# Autodesk Inventor assembly: a shock cartridge
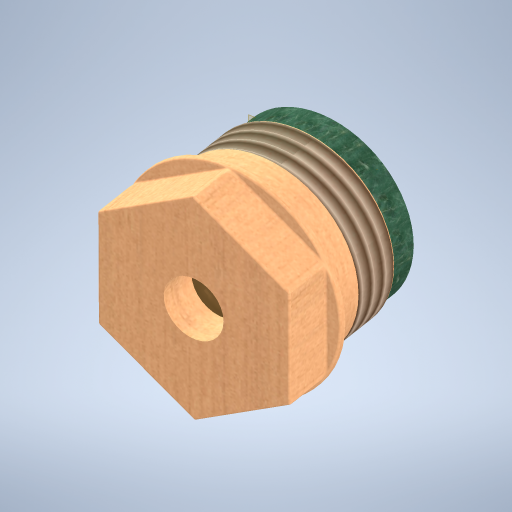
[picture p0: Inventor's stored thumbnail of the model, 512x512]
Saved by Autodesk Inventor 2024 (Build 280153000, 153)
## iProperties
Created: 2023-07-07
Part Number: a shock cartridge
Document SubType Name: Assembly
Designer: birud
Author: birud
## Documents named in this file (5)
- C:\Users\birud\OneDrive\Desktop\Openers\a shock cartridge.iam
- C:\Users\birud\OneDrive\Desktop\Openers\SA Shock Cartridge.ipt
- C:\Users\birud\OneDrive\Desktop\Openers\SA O-Ring-1 final.ipt
- C:\Users\birud\OneDrive\Desktop\Openers\SA Shock Cartridge Spacer.ipt
- C:\Users\birud\OneDrive\Desktop\Openers\SA Shock Cardridge Cover.ipt
## Components (5 placed, 4 different names)
1. SA Shock Cartridge:1 — Mate:1, Mate:2, Mate:3, Rigid:1, Mate:4, Mate:7
2. SA O-Ring-1 final:1 — Mate:1, Mate:2
3. SA Shock Cartridge Spacer:1 — Mate:3, Rigid:1, Mate:5, Mate:6
4. SA Shock Cardridge Cover:1 — Mate:6, Mate:7
5. SA O-Ring-1 final:2 — Mate:4, Mate:5
## Relationships (8: Mate 7, WeldJoint 1)
- Mate:1: SA Shock Cartridge:1 ↔ SA O-Ring-1 final:1
- Mate:2: SA Shock Cartridge:1 ↔ SA O-Ring-1 final:1
- Mate:3: SA Shock Cartridge:1 ↔ SA Shock Cartridge Spacer:1
- Rigid:1 [WeldJoint] (15.875 mm): SA Shock Cartridge:1 ↔ SA Shock Cartridge Spacer:1
- Mate:4: SA Shock Cartridge:1 ↔ SA O-Ring-1 final:2
- Mate:5: SA Shock Cartridge Spacer:1 ↔ SA O-Ring-1 final:2
- Mate:6: SA Shock Cartridge Spacer:1 ↔ SA Shock Cardridge Cover:1
- Mate:7: SA Shock Cartridge:1 ↔ SA Shock Cardridge Cover:1
